# Autodesk Inventor assembly: Mecanismo_base
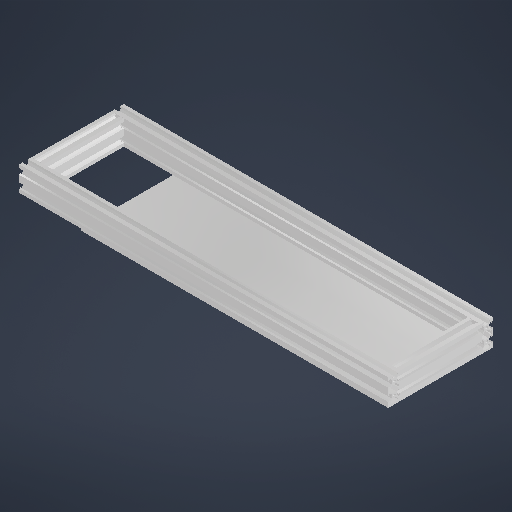
[picture p0: Inventor's stored thumbnail of the model, 512x512]
Saved by Autodesk Inventor 2026 (Build 300175050, 175E)
## iProperties
Created: 2025-10-12
Part Number: Mecanismo_base
Document SubType Name: Assembly
Designer: habbo
Author: habbo
## Documents named in this file (4)
- C:\Users\habbo\OneDrive\Documents\GitHub\Tesis_Mecanismo\CAD\Mecanismo_base_2.iam
- C:\Users\habbo\OneDrive\Documents\GitHub\Tesis_Mecanismo\CAD\Piezas Variadas\V_slots\vslot_2040_130mm.ipt
- C:\Users\habbo\OneDrive\Documents\GitHub\Tesis_Mecanismo\CAD\Piezas Variadas\V_slots\vslot_2040_600mm.ipt
- C:\Users\habbo\OneDrive\Documents\GitHub\Tesis_Mecanismo\CAD\Mecanismo_base_al.ipt
## Components (5 placed, 3 different names)
1. vslot_2040_600mm:1 — Flush:2, Mate:2, Flush:4, Flush:5, Flush:6, Mate:3, Mate:4, Flush:7
2. vslot_2040_130mm:1 — Flush:1, Flush:3, Mate:1, Mate:2, Flush:4, Flush:8
3. vslot_2040_600mm:2 — Flush:1, Flush:2, Flush:3, Mate:1
4. vslot_2040_130mm:2 — Flush:5, Flush:6, Mate:3
5. Mecanismo_base_al:1 — Mate:4, Flush:7, Flush:8
## Relationships (12: Flush 8, Mate 4)
- Flush:1: vslot_2040_130mm:1 ↔ vslot_2040_600mm:2
- Flush:2: vslot_2040_600mm:1 ↔ vslot_2040_600mm:2
- Flush:3: vslot_2040_130mm:1 ↔ vslot_2040_600mm:2
- Mate:1: vslot_2040_130mm:1 ↔ vslot_2040_600mm:2
- Mate:2: vslot_2040_600mm:1 ↔ vslot_2040_130mm:1
- Flush:4: vslot_2040_600mm:1 ↔ vslot_2040_130mm:1
- Flush:5: vslot_2040_600mm:1 ↔ vslot_2040_130mm:2
- Flush:6: vslot_2040_600mm:1 ↔ vslot_2040_130mm:2
- Mate:3: vslot_2040_600mm:1 ↔ vslot_2040_130mm:2
- Mate:4: vslot_2040_600mm:1 ↔ Mecanismo_base_al:1
- Flush:7: vslot_2040_600mm:1 ↔ Mecanismo_base_al:1
- Flush:8: vslot_2040_130mm:1 ↔ Mecanismo_base_al:1
